# Autodesk Inventor assembly: postStandSupport
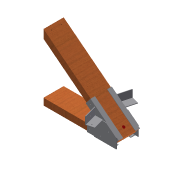
[picture p0: Inventor's stored thumbnail of the model, 180x180]
Saved by Autodesk Inventor 2016 SP2 (Build 200236200, 236)
## iProperties
Created: 2014-08-29
Part Number: postStandSupport
Document SubType Name: Assembly
Designer: Dave
Author: Dave
## Documents named in this file (5)
- C:\Users\krosie\Google Drive\HERA\hera-cad\support\post\postStandSupport.iam
- C:\Users\krosie\Google Drive\HERA\hera-cad\support\post\postStandHoriz.ipt
- C:\Users\krosie\Google Drive\HERA\hera-cad\support\post\postStand37.ipt
- C:\Users\krosie\Google Drive\HERA\hera-cad\support\endcaps\HERA_end_cap_left.iam
- C:\Users\krosie\Google Drive\HERA\hera-cad\support\endcaps\HERA_end_cap_right.iam
## Components (4 placed, 4 different names)
1. HERA_end_cap_left:1 [sub-assembly] — Mate:8, Mate:9, Flush:2, Mate:10, Mate:11, Flush:3, Flush:4, Flush:5
2. postStandHoriz:1 — Mate:8, Mate:9, Flush:2, Mate:12
3. postStand37:1 — Mate:10, Mate:11, Flush:3
4. HERA_end_cap_right:1 [sub-assembly] — Mate:12, Flush:4, Flush:5
## Relationships (9: Mate 5, Flush 4)
- Mate:8: HERA_end_cap_left:1 ↔ postStandHoriz:1
- Mate:9: HERA_end_cap_left:1 ↔ postStandHoriz:1
- Flush:2 (-37 mm): HERA_end_cap_left:1 ↔ postStandHoriz:1
- Mate:10: HERA_end_cap_left:1 ↔ postStand37:1
- Mate:11: HERA_end_cap_left:1 ↔ postStand37:1
- Flush:3: HERA_end_cap_left:1 ↔ postStand37:1
- Mate:12: postStandHoriz:1 ↔ HERA_end_cap_right:1
- Flush:4: HERA_end_cap_left:1 ↔ HERA_end_cap_right:1
- Flush:5: HERA_end_cap_left:1 ↔ HERA_end_cap_right:1
